# Autodesk Inventor assembly: Carril
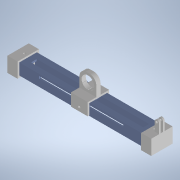
[picture p0: Inventor's stored thumbnail of the model, 180x180]
Saved by Autodesk Inventor 2022 (Build 260153000, 153)
## iProperties
Created: 2022-01-30
Part Number: Carril
Document SubType Name: Assembly
Designer: katha
Author: katha
## Documents named in this file (6)
- C:\Users\katha\OneDrive\Escritorio\Mini_Proyecto_Diseno\Diseno_18012\Modelo_MPD\Carril.iam
- C:\Users\katha\OneDrive\Escritorio\Mini_Proyecto_Diseno\Diseno_18012\Modelo_MPD\Lateral_Carril.ipt
- C:\Users\katha\OneDrive\Escritorio\Mini_Proyecto_Diseno\Diseno_18012\Modelo_MPD\Base_Carril.ipt
- C:\Users\katha\OneDrive\Escritorio\Mini_Proyecto_Diseno\Diseno_18012\Modelo_MPD\Tope_Carril.ipt
- C:\Users\katha\OneDrive\Escritorio\Mini_Proyecto_Diseno\Diseno_18012\Modelo_MPD\Tope_Carril_derecho.ipt
- C:\Users\katha\OneDrive\Escritorio\Mini_Proyecto_Diseno\Diseno_18012\Modelo_MPD\Eje_Carril.ipt
## Components (6 placed, 5 different names)
1. Lateral_Carril:1 — Flush:1, Flush:3, Mate:2, Mate:4, Mate:7, Mate:18
2. Lateral_Carril:2 — Flush:2, Flush:4, Mate:1, Mate:10
3. Base_Carril:1 — Flush:1, Flush:2, Flush:3, Flush:4, Mate:1, Mate:2, Mate:3, Mate:5, Mate:6, Mate:8, Mate:17
4. Tope_Carril:1 — Mate:3, Mate:4, Mate:5
5. Tope_Carril_derecho:1 — Mate:6, Mate:7, Mate:8
6. Eje_Carril:1 — Mate:10, Mate:17, Mate:18
## Relationships (15: Mate 11, Flush 4)
- Flush:1: Lateral_Carril:1 ↔ Base_Carril:1
- Flush:2: Lateral_Carril:2 ↔ Base_Carril:1
- Flush:3: Lateral_Carril:1 ↔ Base_Carril:1
- Flush:4: Lateral_Carril:2 ↔ Base_Carril:1
- Mate:1: Lateral_Carril:2 ↔ Base_Carril:1
- Mate:2: Lateral_Carril:1 ↔ Base_Carril:1
- Mate:3 (0.3 mm): Base_Carril:1 ↔ Tope_Carril:1
- Mate:4: Lateral_Carril:1 ↔ Tope_Carril:1
- Mate:5: Base_Carril:1 ↔ Tope_Carril:1
- Mate:6 (0.3 mm): Base_Carril:1 ↔ Tope_Carril_derecho:1
- Mate:7: Lateral_Carril:1 ↔ Tope_Carril_derecho:1
- Mate:8: Base_Carril:1 ↔ Tope_Carril_derecho:1
- Mate:10 (0.3 mm): Lateral_Carril:2 ↔ Eje_Carril:1
- Mate:17 (0.2 mm): Base_Carril:1 ↔ Eje_Carril:1
- Mate:18 (0.119 mm): Lateral_Carril:1 ↔ Eje_Carril:1
